# Autodesk Inventor assembly: PasekZebaty
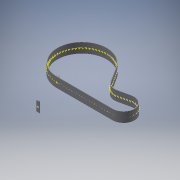
[picture p0: Inventor's stored thumbnail of the model, 180x180]
Saved by Autodesk Inventor 2019 (Build 230136000, 136)
## iProperties
Created: 2020-05-23
Part Number: PasekZebaty
Document SubType Name: Assembly
Designer: estee
Author: estee
## Documents named in this file (3)
- C:\Users\estee\OneDrive\Pulpit\estere\1\MUM\projejt\PasekZebaty.iam
- C:\Users\estee\OneDrive\Pulpit\estere\1\MUM\projejt\PasekZebaty.ipt
- C:\Users\estee\OneDrive\Pulpit\estere\1\MUM\projejt\zab.ipt
## Components (3 placed, 2 different names)
1. PasekZebaty:1 — Mate:1, Flush:1, Mate:2
2. zab:1 — Mate:1, Flush:1, Mate:2
3. zab:2
## Relationships (3: Mate 2, Flush 1)
- Mate:1: PasekZebaty:1 ↔ zab:1
- Flush:1: PasekZebaty:1 ↔ zab:1
- Mate:2: PasekZebaty:1 ↔ zab:1
